# Autodesk Inventor assembly: AKK RS2205 2300KV
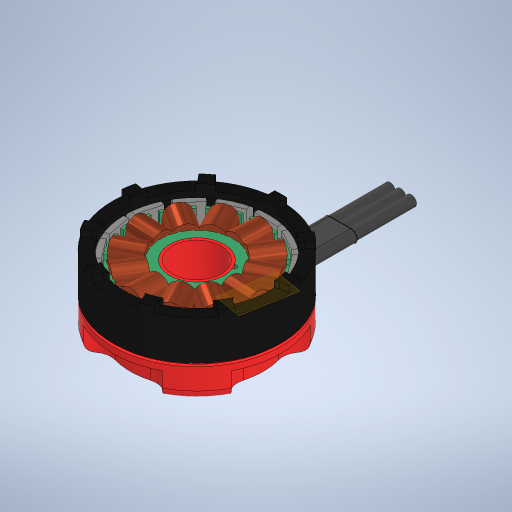
[picture p0: Inventor's stored thumbnail of the model, 512x512]
Saved by Autodesk Inventor 2023.4 (Build 274418000, 418)
## iProperties
Created: 2024-02-02
Part Number: AKK RS2205 2300KV
Document SubType Name: Assembly
Designer: Nathan Cai
Mass: 28.8 g
Surface Area: 85.8074 cm^2
Volume: 4.18383 cm^3
Sending System: Autodesk Inventor 2023
Preprocessor: ST-DEVELOPER v19.2
Title: AKK RS2205 2300KV.stp
Author: Nathan Cai
## Documents named in this file (11)
- E:\Documents\Inventor\Bleep V1.2\AKK RS2205 2300KV\AKK RS2205 2300KV.iam
- E:\Documents\Inventor\Bleep V1.2\AKK RS2205 2300KV\BEARING.ipt
- E:\Documents\Inventor\Bleep V1.2\AKK RS2205 2300KV\STATOR.ipt
- E:\Documents\Inventor\Bleep V1.2\AKK RS2205 2300KV\CAN.ipt
- E:\Documents\Inventor\Bleep V1.2\AKK RS2205 2300KV\SHAFT.ipt
- E:\Documents\Inventor\Bleep V1.2\AKK RS2205 2300KV\98541A111_External Retaining Ring.ipt
- E:\Documents\Inventor\Bleep V1.2\AKK RS2205 2300KV\SPACER.ipt
- E:\Documents\Inventor\Bleep V1.2\AKK RS2205 2300KV\COILS.ipt
- E:\Documents\Inventor\Bleep V1.2\AKK RS2205 2300KV\Magnets.ipt
- E:\Documents\Inventor\Bleep V1.2\AKK RS2205 2300KV\Cable Sleeve.ipt
- E:\Documents\Inventor\Bleep V1.2\AKK RS2205 2300KV\BASE.ipt
## Components (35 placed, 10 different names)
1. BEARING:1
2. BEARING:2
3. STATOR:1 — Mate:1, Flush:1
4. CAN:1
5. SHAFT:1
6. 98541A111_External Retaining Ring:1
7. SPACER:1
8. COILS:1
9. COILS:2
10. COILS:3
11. COILS:4
12. COILS:5
13. COILS:6
14. COILS:7
15. COILS:8
16. COILS:9
17. COILS:10
18. COILS:11
19. COILS:12
20. Magnets:1
21. Magnets:2
22. Magnets:3
23. Magnets:4
24. Magnets:5
25. Magnets:6
26. Magnets:7
27. Magnets:8
28. Magnets:9
29. Magnets:10
30. Magnets:11
31. Magnets:12
32. Magnets:13
33. Magnets:14
34. Cable Sleeve:1
35. BASE:1 — Mate:1, Flush:1
## Relationships (2: Mate 1, Flush 1)
- Mate:1: STATOR:1 ↔ BASE:1
- Flush:1: STATOR:1 ↔ BASE:1
